# Autodesk Inventor assembly: Internal Rear Panel Assembly
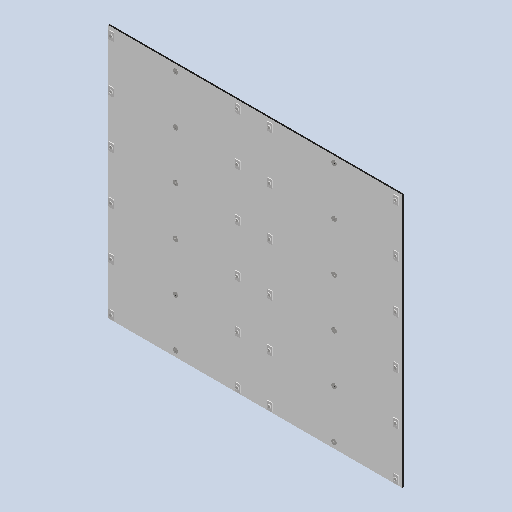
[picture p0: Inventor's stored thumbnail of the model, 512x512]
Saved by Autodesk Inventor 2024 (Build 280153000, 153)
## iProperties
Created: 2024-10-26
Part Number: Internal Rear Panel Assembly
Document SubType Name: Assembly
Designer: Ishaan
Author: Ishaan
## Documents named in this file (4)
- E:\Projects\Axiom--IDEX-3D-Printer\CAD\08 - Side Panelling\Internal Rear Panel Assembly.iam
- E:\Projects\Axiom--IDEX-3D-Printer\CAD\08 - Side Panelling\Rear Internal Side Panel R2.ipt
- E:\Projects\Axiom--IDEX-3D-Printer\CAD\00 - COTS Components\Hardware\Low Profile M5x8.ipt
- E:\Projects\Axiom--IDEX-3D-Printer\CAD\00 - COTS Components\Hardware\M5 T SLOT NUT.ipt
## Components (73 placed, 3 different names)
1. Rear Internal Side Panel R2:1 — Insert:1, Insert:2, Insert:3, Insert:4, Angle:1, Insert:5, Angle:2, Insert:6, Angle:3
2. Low Profile M5x8:1 — Insert:1
3. Low Profile M5x8:2
4. Low Profile M5x8:3
5. Low Profile M5x8:4
6. Low Profile M5x8:5
7. Low Profile M5x8:6
8. Low Profile M5x8:7
9. Low Profile M5x8:8
10. Low Profile M5x8:9
11. Low Profile M5x8:10
12. Low Profile M5x8:11
13. Low Profile M5x8:12
14. Low Profile M5x8:13 — Insert:2
15. Low Profile M5x8:14
16. Low Profile M5x8:15
17. Low Profile M5x8:16
18. Low Profile M5x8:17
19. Low Profile M5x8:18
20. Low Profile M5x8:19
21. Low Profile M5x8:20
22. Low Profile M5x8:21
23. Low Profile M5x8:22
24. Low Profile M5x8:23
25. Low Profile M5x8:24
26. Low Profile M5x8:25 — Insert:3
27. Low Profile M5x8:26
28. Low Profile M5x8:27
29. Low Profile M5x8:28
30. Low Profile M5x8:29
31. Low Profile M5x8:30
32. Low Profile M5x8:31
33. Low Profile M5x8:32
34. Low Profile M5x8:33
35. Low Profile M5x8:34
36. Low Profile M5x8:35
37. Low Profile M5x8:36
38. M5 T SLOT NUT:1 — Insert:4, Angle:1
39. M5 T SLOT NUT:2
40. M5 T SLOT NUT:3
41. M5 T SLOT NUT:4
42. M5 T SLOT NUT:5
43. M5 T SLOT NUT:6
44. M5 T SLOT NUT:7
45. M5 T SLOT NUT:8
46. M5 T SLOT NUT:9
47. M5 T SLOT NUT:10
48. M5 T SLOT NUT:11
49. M5 T SLOT NUT:12
50. M5 T SLOT NUT:13 — Insert:5, Angle:2
51. M5 T SLOT NUT:14
52. M5 T SLOT NUT:15
53. M5 T SLOT NUT:16
54. M5 T SLOT NUT:17
55. M5 T SLOT NUT:18
56. M5 T SLOT NUT:19
57. M5 T SLOT NUT:20
58. M5 T SLOT NUT:21
59. M5 T SLOT NUT:22
60. M5 T SLOT NUT:23
61. M5 T SLOT NUT:24
62. M5 T SLOT NUT:25 — Insert:6, Angle:3
63. M5 T SLOT NUT:26
64. M5 T SLOT NUT:27
65. M5 T SLOT NUT:28
66. M5 T SLOT NUT:29
67. M5 T SLOT NUT:30
68. M5 T SLOT NUT:31
69. M5 T SLOT NUT:32
70. M5 T SLOT NUT:33
71. M5 T SLOT NUT:34
72. M5 T SLOT NUT:35
73. M5 T SLOT NUT:36
## Component patterns: (12 elements, first: Low Profile M5x8:1), (12 elements, first: Low Profile M5x8:13), (12 elements, first: Low Profile M5x8:25), (12 elements, first: M5 T SLOT NUT:1), (12 elements, first: M5 T SLOT NUT:13), (12 elements, first: M5 T SLOT NUT:25)
## Relationships (9: Insert 6, Angle 3)
- Insert:1: Rear Internal Side Panel R2:1 ↔ Low Profile M5x8:1
- Insert:2: Rear Internal Side Panel R2:1 ↔ Low Profile M5x8:13
- Insert:3: Rear Internal Side Panel R2:1 ↔ Low Profile M5x8:25
- Insert:4 (2 mm): Rear Internal Side Panel R2:1 ↔ M5 T SLOT NUT:1
- Angle:1 (0 deg): Rear Internal Side Panel R2:1 ↔ M5 T SLOT NUT:1
- Insert:5 (2 mm): Rear Internal Side Panel R2:1 ↔ M5 T SLOT NUT:13
- Angle:2 (0 deg): Rear Internal Side Panel R2:1 ↔ M5 T SLOT NUT:13
- Insert:6 (2 mm): Rear Internal Side Panel R2:1 ↔ M5 T SLOT NUT:25
- Angle:3 (0 deg): Rear Internal Side Panel R2:1 ↔ M5 T SLOT NUT:25
